# Autodesk Inventor assembly: FrontGearboxAssembly_MIR
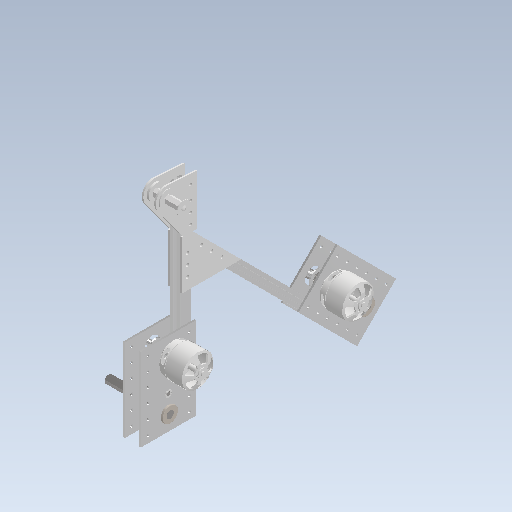
[picture p0: Inventor's stored thumbnail of the model, 512x512]
Saved by Autodesk Inventor 2023 (Build 270158000, 158)
## iProperties
Created: 2023-02-14
Part Number: FrontGearboxAssembly_MIR
Document SubType Name: Assembly
Designer: Dave
Author: Dave
## Documents named in this file (7)
- C:\Users\Dave\Documents\GitHub\BehrendURCMechanical\CAD\Chassis\GearBox\Final Gears and Assemblies\FrontGearboxAssembly_MIR.iam
- C:\Users\Dave\Documents\GitHub\BehrendURCMechanical\CAD\Chassis\GearBox\Final Gears and Assemblies\Gearbox Assembly_MIR.iam
- C:\Users\Dave\Documents\GitHub\BehrendURCMechanical\CAD\Chassis\CH-1-01-FrontKneeJoint_MIR.ipt
- C:\Users\Dave\Documents\GitHub\BehrendURCMechanical\CAD\Chassis\HipJoint_MIR.iam
- C:\Users\Dave\Documents\GitHub\BehrendURCMechanical\CAD\Chassis\CH-1-01-20x20 Channel\CH-1-01-20x20 Channel-437.ipt
- C:\Users\Dave\Documents\GitHub\BehrendURCMechanical\CAD\Chassis\CH-1-01-20x20 Channel.ipt
- C:\Users\Dave\Documents\GitHub\BehrendURCMechanical\CAD\Chassis\CH-1-01-20x20 Channel\CH-1-01-20x20 Channel-372.ipt
## Components (7 placed, 5 different names)
1. Gearbox Assembly_MIR:1 [sub-assembly] — Mate:15, Flush:13, Tangent:1, Angle:1, Angle:2, Flush:1, Flush:19, Flush:18
2. Gearbox Assembly_MIR:2 [sub-assembly] — Angle:2, Flush:1, Flush:21
3. CH-1-01-FrontKneeJoint_MIR:1 — Flush:12, Flush:11, Mate:19
4. HipJoint_MIR:1 [sub-assembly] — Mate:18, Tangent:2, Mate:22
5. CH-1-01-FrontKneeJoint_MIR:2 — Mate:18, Flush:12, Flush:11, Flush:14, Flush:20
6. CH-1-01-20x20 Channel-437:1 — Flush:21, Flush:14, Mate:19, Flush:17
7. CH-1-01-20x20 Channel-372:2 — Flush:20, Tangent:2, Flush:19, Flush:18, Mate:22, Flush:17
## Relationships (18: Flush 11, Mate 3, Tangent 2, Angle 2)
- Mate:15 [Flush]: Gearbox Assembly_MIR:1
- Flush:13: Gearbox Assembly_MIR:1
- Tangent:1: Gearbox Assembly_MIR:1
- Angle:1 (90 deg): Gearbox Assembly_MIR:1
- Angle:2 (-45 deg): Gearbox Assembly_MIR:1 ↔ Gearbox Assembly_MIR:2
- Flush:1: Gearbox Assembly_MIR:1 ↔ Gearbox Assembly_MIR:2
- Mate:18: HipJoint_MIR:1 ↔ CH-1-01-FrontKneeJoint_MIR:2
- Flush:12: CH-1-01-FrontKneeJoint_MIR:1 ↔ CH-1-01-FrontKneeJoint_MIR:2
- Flush:11: CH-1-01-FrontKneeJoint_MIR:1 ↔ CH-1-01-FrontKneeJoint_MIR:2
- Flush:21 (-2.6924 mm): Gearbox Assembly_MIR:2 ↔ CH-1-01-20x20 Channel-437:1
- Flush:14: CH-1-01-FrontKneeJoint_MIR:2 ↔ CH-1-01-20x20 Channel-437:1
- Mate:19: CH-1-01-FrontKneeJoint_MIR:1 ↔ CH-1-01-20x20 Channel-437:1
- Flush:20: CH-1-01-FrontKneeJoint_MIR:2 ↔ CH-1-01-20x20 Channel-372:2
- Tangent:2: HipJoint_MIR:1 ↔ CH-1-01-20x20 Channel-372:2
- Flush:19 (2.6924 mm): Gearbox Assembly_MIR:1 ↔ CH-1-01-20x20 Channel-372:2
- Flush:18: Gearbox Assembly_MIR:1 ↔ CH-1-01-20x20 Channel-372:2
- Mate:22: HipJoint_MIR:1 ↔ CH-1-01-20x20 Channel-372:2
- Flush:17: CH-1-01-20x20 Channel-437:1 ↔ CH-1-01-20x20 Channel-372:2
